# Autodesk Inventor assembly: DCSM Leg Assembly
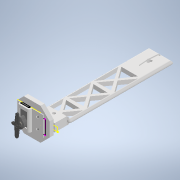
[picture p0: Inventor's stored thumbnail of the model, 180x180]
Saved by Autodesk Inventor 2020 (Build 240168000, 168)
## iProperties
Created: 2020-03-18
Part Number: DCSM Leg Assembly
Document SubType Name: Assembly
Designer: varun
Author: varun
## Documents named in this file (3)
- C:\Users\varun\Desktop\ServoArm\DCSM Leg Assembly.iam
- C:\Users\varun\Desktop\ServoArm\DCSM Servo Assembly.iam
- C:\Users\varun\Desktop\ServoArm\First Leg.ipt
## Components (2 placed, 2 different names)
1. DCSM Servo Assembly:1 [sub-assembly] — Mate:1, Mate:2, Mate:3
2. First Leg:1 — Mate:1, Mate:2, Mate:3
## Relationships (3: Mate 3)
- Mate:1: DCSM Servo Assembly:1 ↔ First Leg:1
- Mate:2: DCSM Servo Assembly:1 ↔ First Leg:1
- Mate:3: DCSM Servo Assembly:1 ↔ First Leg:1
